# Autodesk Inventor assembly: slimV1_mockup
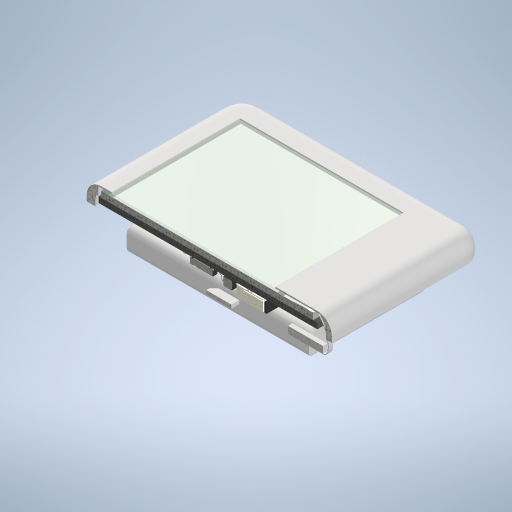
[picture p0: Inventor's stored thumbnail of the model, 512x512]
Saved by Autodesk Inventor 2023 (Build 270158000, 158)
## iProperties
Created: 2023-03-12
Part Number: slimV1_mockup
Document SubType Name: Assembly
Designer: nigel
Author: nigel
## Documents named in this file (5)
- D:\NIGEL\Documents\GitHub\Watchy-CAD\CAD\Cases\SlimTouchscreenV1\slimV1_mockup.iam
- D:\NIGEL\Documents\GitHub\Watchy-CAD\CAD\Cases\SlimTouchscreenV1\SLIM_TC_ASSEMBLED_V1.iam
- D:\NIGEL\Documents\GitHub\Watchy-CAD\CAD\Cases\SlimTouchscreenV1\case_mockup2.ipt
- D:\NIGEL\Documents\GitHub\Watchy-CAD\CAD\Base Model\Battery_402535.ipt
- D:\NIGEL\Documents\GitHub\Watchy-CAD\CAD\Cases\SlimTouchscreenV1\Button.ipt
## Components (7 placed, 4 different names)
1. SLIM_TC_ASSEMBLED_V1:1 [sub-assembly] — Flush:2, Mate:2, Mate:3
2. case_mockup2:1 — Flush:2, Mate:2, Mate:3, Mate:4, Mate:5, Mate:6, Mate:7, Mate:8, Mate:9, Mate:10, Mate:11
3. Battery_402535:1
4. Button:1 — Mate:5, Mate:8
5. Button:2 — Mate:4, Mate:9
6. Button:3 — Mate:6, Mate:11
7. Button:4 — Mate:7, Mate:10
## Relationships (11: Mate 10, Flush 1)
- Flush:2: SLIM_TC_ASSEMBLED_V1:1 ↔ case_mockup2:1
- Mate:2: SLIM_TC_ASSEMBLED_V1:1 ↔ case_mockup2:1
- Mate:3: SLIM_TC_ASSEMBLED_V1:1 ↔ case_mockup2:1
- Mate:4: case_mockup2:1 ↔ Button:2
- Mate:5: case_mockup2:1 ↔ Button:1
- Mate:6: case_mockup2:1 ↔ Button:3
- Mate:7: case_mockup2:1 ↔ Button:4
- Mate:8: case_mockup2:1 ↔ Button:1
- Mate:9: case_mockup2:1 ↔ Button:2
- Mate:10: case_mockup2:1 ↔ Button:4
- Mate:11: case_mockup2:1 ↔ Button:3
